# Autodesk Inventor assembly: 8 Pin female
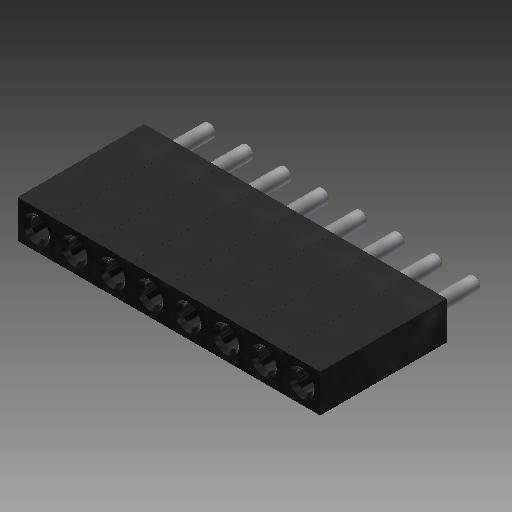
[picture p0: Inventor's stored thumbnail of the model, 512x512]
Saved by Autodesk Inventor 2017 (Build 210142000, 142)
## iProperties
Created: 2016-08-05
Part Number: 8 Pin female
Document SubType Name: Assembly
Designer: ge937963
Author: ge937963
## Documents named in this file (2)
- P:\allusers\Diagnostics\Inventor Files\3dPrintedPCR\8 Pin female.iam
- P:\allusers\Diagnostics\Inventor Files\3dPrintedPCR\Female Header.ipt
## Components (8 placed, 1 different names)
1. Female Header:1 — Flush:1, Flush:2, Mate:1
2. Female Header:2 — Flush:1, Flush:2, Mate:1, Flush:3, Flush:9, Mate:2
3. Female Header:3 — Flush:3, Flush:4, Flush:9, Flush:10, Mate:2, Mate:3
4. Female Header:4 — Flush:4, Flush:5, Flush:10, Flush:11, Mate:3, Mate:4
5. Female Header:5 — Flush:5, Flush:6, Flush:11, Flush:12, Mate:4, Mate:5
6. Female Header:6 — Flush:6, Flush:7, Flush:12, Flush:13, Mate:5, Mate:6
7. Female Header:7 — Flush:7, Flush:8, Flush:13, Flush:14, Mate:6, Mate:7
8. Female Header:8 — Flush:8, Flush:14, Mate:7
## Relationships (21: Flush 14, Mate 7)
- Flush:1: Female Header:1 ↔ Female Header:2
- Flush:2: Female Header:1 ↔ Female Header:2
- Mate:1: Female Header:1 ↔ Female Header:2
- Flush:3: Female Header:2 ↔ Female Header:3
- Flush:4: Female Header:3 ↔ Female Header:4
- Flush:5: Female Header:4 ↔ Female Header:5
- Flush:6: Female Header:5 ↔ Female Header:6
- Flush:7: Female Header:6 ↔ Female Header:7
- Flush:8: Female Header:7 ↔ Female Header:8
- Flush:9: Female Header:2 ↔ Female Header:3
- Flush:10: Female Header:3 ↔ Female Header:4
- Flush:11: Female Header:4 ↔ Female Header:5
- Flush:12: Female Header:5 ↔ Female Header:6
- Flush:13: Female Header:6 ↔ Female Header:7
- Flush:14: Female Header:7 ↔ Female Header:8
- Mate:2: Female Header:2 ↔ Female Header:3
- Mate:3: Female Header:3 ↔ Female Header:4
- Mate:4: Female Header:4 ↔ Female Header:5
- Mate:5: Female Header:5 ↔ Female Header:6
- Mate:6: Female Header:6 ↔ Female Header:7
- Mate:7: Female Header:7 ↔ Female Header:8
